# Autodesk Inventor assembly: borneras
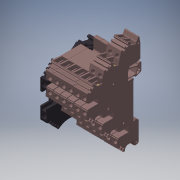
[picture p0: Inventor's stored thumbnail of the model, 180x180]
Saved by Autodesk Inventor 2017 (Build 210142000, 142)
## iProperties
Created: 2017-10-02
Part Number: borneras
Document SubType Name: Assembly
Designer: Alejandro
Author: Alejandro
## Documents named in this file (4)
- C:\Users\user\Documents\Universidad - Mecatrónica\Semestre 9\Diseño Mecatrónico\Parcial 1\Piezas\Borneras juntas\borneras.iam
- C:\Users\user\Documents\Universidad - Mecatrónica\Semestre 9\Diseño Mecatrónico\Parcial 1\Piezas\65550016-9-58162\58162.ipt
- C:\Users\user\Documents\Universidad - Mecatrónica\Semestre 9\Diseño Mecatrónico\Parcial 1\Piezas\65551450-9-58161\58161.ipt
- C:\Users\user\Documents\Universidad - Mecatrónica\Semestre 9\Diseño Mecatrónico\Parcial 1\Piezas\65553036-9-57938\57938.ipt
## Components (7 placed, 3 different names)
1. 58162:1 — Mate:1, Mate:5
2. 58162:2 — Mate:1, Mate:2
3. 58162:3 — Mate:2, Mate:3
4. 58162:4 — Mate:3, Mate:4
5. 58161:1 — Mate:4, Mate:6
6. 57938:1 — Mate:5
7. 58161:2 — Mate:6
## Relationships (6: Mate 6)
- Mate:1: 58162:1 ↔ 58162:2
- Mate:2: 58162:2 ↔ 58162:3
- Mate:3: 58162:3 ↔ 58162:4
- Mate:4: 58162:4 ↔ 58161:1
- Mate:5: 58162:1 ↔ 57938:1
- Mate:6: 58161:1 ↔ 58161:2
